# Autodesk Inventor assembly: mousetrap19
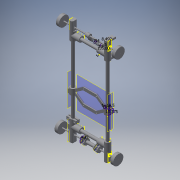
[picture p0: Inventor's stored thumbnail of the model, 180x180]
Saved by Autodesk Inventor 2018 (Build 220112000, 112)
## iProperties
Created: 2018-11-24
Part Number: mousetrap19
Document SubType Name: Assembly
Designer: Prakash
Author: Prakash
## Documents named in this file (16)
- C:\Users\Prakash\Documents\Inventor\Mousetrap 2018\mousetrap19.iam
- C:\Users\Prakash\Documents\Inventor\Mousetrap 2018\LBChassis.ipt
- C:\Users\Prakash\Documents\Inventor\Mousetrap 2018\LFChassis.ipt
- C:\Users\Prakash\Documents\Inventor\Mousetrap 2018\RBChassiss.ipt
- C:\Users\Prakash\Documents\Inventor\Mousetrap 2018\RFChassis.ipt
- C:\Users\Prakash\Documents\Inventor\Mousetrap 2018\LongCF.ipt
- C:\Users\Prakash\Documents\Inventor\Mousetrap 2018\ShortCF.ipt
- C:\Users\Prakash\Documents\Inventor\Mousetrap 2018\Axles.ipt
- C:\Users\Prakash\Documents\Inventor\Mousetrap 2018\spindles.ipt
- C:\Users\Prakash\Documents\Inventor\Mousetrap 2018\93355A310_LOW-STRENGTH STL HEX CPLG NUT.ipt
- C:\Users\Prakash\Documents\Inventor\Mousetrap 2018\wingnut.ipt
- C:\Users\Prakash\Documents\Inventor\Mousetrap 2018\springStub.ipt
- C:\Users\Prakash\Documents\Inventor\Mousetrap 2018\9434K152_MUSIC WIRE PRECISION COMPRESSION SPRING.ipt
- C:\Users\Prakash\Documents\Inventor\Mousetrap 2018\mousetrapMount.ipt
- C:\Users\Prakash\Documents\Inventor\Mousetrap 2018\wheels.ipt
- C:\Users\Prakash\Documents\Inventor\Mousetrap 2018\clampCap.ipt
## Components (21 placed, 15 different names)
1. LBChassis:1 — Mate:1, Mate:2, Mate:11, Mate:15
2. LFChassis:1 — Mate:3, Mate:4, Mate:9, Mate:21, Mate:22, Mate:24
3. RBChassiss:1 — Mate:5, Mate:8, Mate:12, Mate:13, Mate:17, Mate:33, Angle:3
4. RFChassis:1 — Mate:6, Mate:7, Mate:10, Mate:14, Mate:16
5. LongCF:1 — Mate:5, Mate:6, Mate:7, Mate:8, Mate:25, Mate:32
6. LongCF:2 — Mate:1, Mate:2, Mate:3, Mate:4
7. ShortCF:1 — Mate:11, Mate:12, Mate:13, Mate:15
8. ShortCF:2 — Mate:9, Mate:10, Mate:14
9. Axles:1 — Mate:16, Mate:20, Mate:28, Mate:29, Mate:30, Flush:2
10. Axles:2 — Mate:17, Mate:18, Mate:26, Mate:27, Flush:3, Mate:31
11. spindles:1 — Mate:18
12. 93355A310_LOW-STRENGTH STL HEX CPLG NUT:1 — Mate:19, Angle:1, Flush:1, Mate:20
13. wingnut:1 — Mate:19, Angle:1, Flush:1
14. springStub:1 — Mate:21, Mate:22, Mate:23
15. 9434K152_MUSIC WIRE PRECISION COMPRESSION SPRING:1 — Mate:23, Mate:24
16. mousetrapMount:1 — Mate:25, Angle:2
17. wheels:1 — Mate:26, Mate:27
18. wheels:2 — Mate:30, Flush:2
19. wheels:3 — Flush:3, Mate:31
20. wheels:4 — Mate:28, Mate:29
21. clampCap:1 — Mate:32, Mate:33, Angle:3
## Relationships (39: Mate 33, Angle 3, Flush 3)
- Mate:1: LBChassis:1 ↔ LongCF:2
- Mate:2: LBChassis:1 ↔ LongCF:2
- Mate:3: LFChassis:1 ↔ LongCF:2
- Mate:4: LFChassis:1 ↔ LongCF:2
- Mate:5: RBChassiss:1 ↔ LongCF:1
- Mate:6: RFChassis:1 ↔ LongCF:1
- Mate:7: RFChassis:1 ↔ LongCF:1
- Mate:8: RBChassiss:1 ↔ LongCF:1
- Mate:9: LFChassis:1 ↔ ShortCF:2
- Mate:10: RFChassis:1 ↔ ShortCF:2
- Mate:11: LBChassis:1 ↔ ShortCF:1
- Mate:12: RBChassiss:1 ↔ ShortCF:1
- Mate:13: RBChassiss:1 ↔ ShortCF:1
- Mate:14: RFChassis:1 ↔ ShortCF:2
- Mate:15: LBChassis:1 ↔ ShortCF:1
- Mate:16: RFChassis:1 ↔ Axles:1
- Mate:17: RBChassiss:1 ↔ Axles:2
- Mate:18: Axles:2 ↔ spindles:1
- Mate:19: 93355A310_LOW-STRENGTH STL HEX CPLG NUT:1 ↔ wingnut:1
- Angle:1 (0 deg): 93355A310_LOW-STRENGTH STL HEX CPLG NUT:1 ↔ wingnut:1
- Flush:1: 93355A310_LOW-STRENGTH STL HEX CPLG NUT:1 ↔ wingnut:1
- Mate:20: Axles:1 ↔ 93355A310_LOW-STRENGTH STL HEX CPLG NUT:1
- Mate:21: LFChassis:1 ↔ springStub:1
- Mate:22: LFChassis:1 ↔ springStub:1
- Mate:23: springStub:1 ↔ 9434K152_MUSIC WIRE PRECISION COMPRESSION SPRING:1
- Mate:24: LFChassis:1 ↔ 9434K152_MUSIC WIRE PRECISION COMPRESSION SPRING:1
- Mate:25: LongCF:1 ↔ mousetrapMount:1
- Angle:2 (0 deg): mousetrapMount:1
- Mate:26: Axles:2 ↔ wheels:1
- Mate:27: Axles:2 ↔ wheels:1
- Mate:28: Axles:1 ↔ wheels:4
- Mate:29: Axles:1 ↔ wheels:4
- Mate:30: Axles:1 ↔ wheels:2
- Flush:2: Axles:1 ↔ wheels:2
- Flush:3: Axles:2 ↔ wheels:3
- Mate:31: Axles:2 ↔ wheels:3
- Mate:32: LongCF:1 ↔ clampCap:1
- Mate:33: RBChassiss:1 ↔ clampCap:1
- Angle:3 (0 deg): RBChassiss:1 ↔ clampCap:1
